# Autodesk Inventor assembly: Arc Reactor
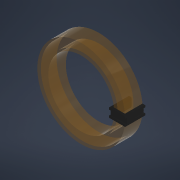
[picture p0: Inventor's stored thumbnail of the model, 180x180]
Saved by Autodesk Inventor 2022.4 (Build 264492010, 492A)
## iProperties
Created: 2023-10-10
Part Number: Arc Reactor
Document SubType Name: Assembly
Designer: Harsh
Author: Harsh
## Documents named in this file (3)
- C:\Users\Harsh\OneDrive\Documents\Side Porjects\Iron Man Arc Reactor\Arc Reactor.iam
- C:\Users\Harsh\OneDrive\Documents\Side Porjects\Iron Man Arc Reactor\Cylinder Beam.ipt
- C:\Users\Harsh\OneDrive\Documents\Side Porjects\Iron Man Arc Reactor\Coils.ipt
## Components (2 placed, 2 different names)
1. Cylinder Beam:1 — Flush:1
2. Coils:1 — Flush:1
## Relationships (1: Flush 1)
- Flush:1: Cylinder Beam:1 ↔ Coils:1
